# Autodesk Inventor assembly: Cart assembly
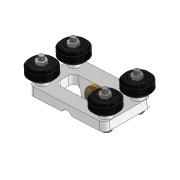
[picture p0: Inventor's stored thumbnail of the model, 180x180]
Saved by Autodesk Inventor 2020 (Build 240168000, 168)
## iProperties
Created: 2020-12-15
Part Number: Cart assembly
Document SubType Name: Assembly
Designer: ferrerx
Author: ferrerx
## Documents named in this file (8)
- C:\Users\ferrerx\Desktop\Prieto-Godino Lab\Drosophila Larvae Behavioural Device\Device design V3\Inventor Assembly\Cart assembly.iam
- C:\Users\ferrerx\Desktop\Prieto-Godino Lab\Drosophila Larvae Behavioural Device\Device design V3\Inventor Assembly\Cart.ipt
- C:\Users\ferrerx\Desktop\Prieto-Godino Lab\Drosophila Larvae Behavioural Device\Device design V3\Inventor Assembly\cart_spacer.ipt
- C:\Users\ferrerx\Desktop\Prieto-Godino Lab\Drosophila Larvae Behavioural Device\Device design V3\Inventor Assembly\guide wheel.ipt
- C:\Users\ferrerx\Desktop\Prieto-Godino Lab\Drosophila Larvae Behavioural Device\Device design V3\Inventor Assembly\lead screw nut.ipt
- C:\Users\ferrerx\Documents\Inventor\Content Center Files\R2020\en-US\AS 1427(05)\AS 1427 - M3 x 20(5) II.ipt
- C:\Users\ferrerx\Documents\Inventor\Content Center Files\R2020\en-US\AS 1427(10)\AS 1427 - M5 x 30(7).ipt
- C:\Users\ferrerx\Documents\Inventor\Content Center Files\R2020\en-US\BS 4183(1)\BS 4183 - M5(1).ipt
## Components (22 placed, 7 different names)
1. Cart:1 — Mate:1, Mate:2, Mate:3, Mate:4, Mate:5, Mate:6, Mate:7, Mate:8, Mate:9, Mate:10, Mate:11, Mate:12, Mate:13, Mate:14, Mate:15, Mate:22, Mate:23, Mate:24, Mate:25, Mate:26, Mate:27, Mate:28, Mate:29, Mate:30, Mate:31, Mate:32, Mate:33, Mate:34
2. cart_spacer:1 — Mate:4, Mate:8, Mate:16
3. cart_spacer:2 — Mate:5, Mate:9, Mate:18
4. cart_spacer:3 — Mate:6, Mate:10, Mate:19
5. cart_spacer:4 — Mate:7, Mate:11, Mate:17
6. guide wheel:1 — Mate:15, Mate:18, Mate:42
7. guide wheel:2 — Mate:14, Mate:17, Mate:40
8. guide wheel:3 — Mate:13, Mate:16, Mate:41
9. guide wheel:4 — Mate:12, Mate:19, Mate:39
10. lead screw nut:1 — Mate:1, Mate:2, Mate:3, Mate:20, Mate:21
11. AS 1427 H - Metric M3 x 20:1 — Mate:20
12. AS 1427 H - Metric M3 x 20:2 — Mate:21, Mate:22
13. AS 1427 H - Metric M3 x 20:3 — Mate:23, Mate:26
14. AS 1427 H - Metric M3 x 20:4 — Mate:24, Mate:25
15. AS 1427 (8) - Metric M5 x 30:1 — Mate:27, Mate:28, Mate:35
16. AS 1427 (8) - Metric M5 x 30:2 — Mate:29, Mate:34, Mate:36
17. AS 1427 (8) - Metric M5 x 30:3 — Mate:30, Mate:32, Mate:37
18. AS 1427 (8) - Metric M5 x 30:4 — Mate:31, Mate:33, Mate:38
19. BS 4183 - Metric M5:1 — Mate:36, Mate:41
20. BS 4183 - Metric M5:2 — Mate:35, Mate:40
21. BS 4183 - Metric M5:3 — Mate:38, Mate:42
22. BS 4183 - Metric M5:4 — Mate:37, Mate:39
## Relationships (42: Mate 42)
- Mate:1: Cart:1 ↔ lead screw nut:1
- Mate:2: Cart:1 ↔ lead screw nut:1
- Mate:3: Cart:1 ↔ lead screw nut:1
- Mate:4: Cart:1 ↔ cart_spacer:1
- Mate:5: Cart:1 ↔ cart_spacer:2
- Mate:6: Cart:1 ↔ cart_spacer:3
- Mate:7: Cart:1 ↔ cart_spacer:4
- Mate:8: Cart:1 ↔ cart_spacer:1
- Mate:9: Cart:1 ↔ cart_spacer:2
- Mate:10: Cart:1 ↔ cart_spacer:3
- Mate:11: Cart:1 ↔ cart_spacer:4
- Mate:12: Cart:1 ↔ guide wheel:4
- Mate:13: Cart:1 ↔ guide wheel:3
- Mate:14: Cart:1 ↔ guide wheel:2
- Mate:15: Cart:1 ↔ guide wheel:1
- Mate:16: cart_spacer:1 ↔ guide wheel:3
- Mate:17: cart_spacer:4 ↔ guide wheel:2
- Mate:18: cart_spacer:2 ↔ guide wheel:1
- Mate:19: cart_spacer:3 ↔ guide wheel:4
- Mate:20: lead screw nut:1 ↔ AS 1427 H - Metric M3 x 20:1
- Mate:21: lead screw nut:1 ↔ AS 1427 H - Metric M3 x 20:2
- Mate:22: Cart:1 ↔ AS 1427 H - Metric M3 x 20:2
- Mate:23: Cart:1 ↔ AS 1427 H - Metric M3 x 20:3
- Mate:24: Cart:1 ↔ AS 1427 H - Metric M3 x 20:4
- Mate:25: Cart:1 ↔ AS 1427 H - Metric M3 x 20:4
- Mate:26: Cart:1 ↔ AS 1427 H - Metric M3 x 20:3
- Mate:27: Cart:1 ↔ AS 1427 (8) - Metric M5 x 30:1
- Mate:28: Cart:1 ↔ AS 1427 (8) - Metric M5 x 30:1
- Mate:29: Cart:1 ↔ AS 1427 (8) - Metric M5 x 30:2
- Mate:30: Cart:1 ↔ AS 1427 (8) - Metric M5 x 30:3
- Mate:31: Cart:1 ↔ AS 1427 (8) - Metric M5 x 30:4
- Mate:32: Cart:1 ↔ AS 1427 (8) - Metric M5 x 30:3
- Mate:33: Cart:1 ↔ AS 1427 (8) - Metric M5 x 30:4
- Mate:34: Cart:1 ↔ AS 1427 (8) - Metric M5 x 30:2
- Mate:35: AS 1427 (8) - Metric M5 x 30:1 ↔ BS 4183 - Metric M5:2
- Mate:36: AS 1427 (8) - Metric M5 x 30:2 ↔ BS 4183 - Metric M5:1
- Mate:37: AS 1427 (8) - Metric M5 x 30:3 ↔ BS 4183 - Metric M5:4
- Mate:38: AS 1427 (8) - Metric M5 x 30:4 ↔ BS 4183 - Metric M5:3
- Mate:39: guide wheel:4 ↔ BS 4183 - Metric M5:4
- Mate:40: guide wheel:2 ↔ BS 4183 - Metric M5:2
- Mate:41: guide wheel:3 ↔ BS 4183 - Metric M5:1
- Mate:42: guide wheel:1 ↔ BS 4183 - Metric M5:3
